# Autodesk Inventor assembly: podwojne koło zebate
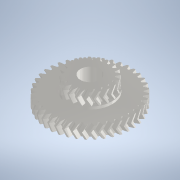
[picture p0: Inventor's stored thumbnail of the model, 180x180]
Saved by Autodesk Inventor 2021 (Build 250183000, 183)
## iProperties
Created: 2021-06-27
Part Number: podwojne koło zebate
Document SubType Name: Assembly
Designer: Łukasz
Author: Łukasz
## Documents named in this file (3)
- E:\GITHUB_Czołg\Szybki-Czolg-antyRadziecki\koła zębate\Design Accelerator\podwojne koło zebate.iam
- E:\GITHUB_Czołg\Szybki-Czolg-antyRadziecki\koła zębate\Design Accelerator\inny set zebow\Design Accelerator\Spur Gear21.ipt
- E:\GITHUB_Czołg\Szybki-Czolg-antyRadziecki\koła zębate\Design Accelerator\inny set zebow\Design Accelerator\Spur Gear11.ipt
## Components (2 placed, 2 different names)
1. Spur Gear2:1 — Rigid:1
2. Spur Gear1:1 — Rigid:1
## Relationships (1: WeldJoint 1)
- Rigid:1 [WeldJoint]: Spur Gear2:1 ↔ Spur Gear1:1
